# Autodesk Inventor assembly: Coil_Of_Wire
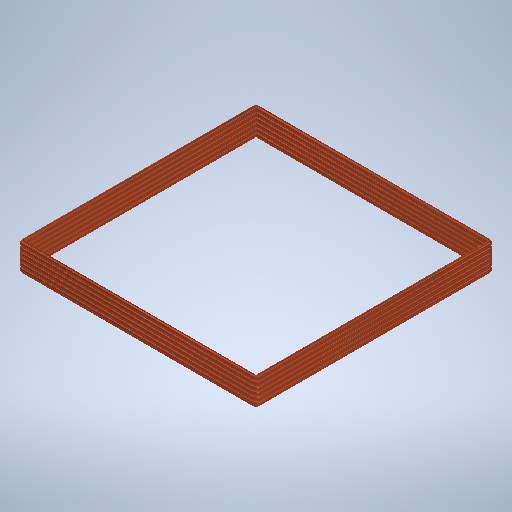
[picture p0: Inventor's stored thumbnail of the model, 512x512]
Saved by Autodesk Inventor 2025 (Build 290162010, 162A)
## iProperties
Created: 2024-10-04
Part Number: Coil_Of_Wire
Document SubType Name: Assembly
Designer: Tom
Author: Tom
## Documents named in this file (2)
- C:\Users\Tom\Documents\Inventor\Mobility\Additional_Building\Coil_Of_Wire.iam
- C:\Users\Tom\Documents\Inventor\Mobility\Additional_Building\Coil_Of_Wire.ipt
## Components (6 placed, 1 different names)
1. Coil_Of_Wire:1 — Flush:1, Flush:2, Flush:3
2. Coil_Of_Wire:2
3. Coil_Of_Wire:3
4. Coil_Of_Wire:4
5. Coil_Of_Wire:5
6. Coil_Of_Wire:6
## Component patterns: (6 elements, first: Coil_Of_Wire:1)
## Relationships (3: Flush 3)
- Flush:1: Coil_Of_Wire:1
- Flush:2: Coil_Of_Wire:1
- Flush:3: Coil_Of_Wire:1
